# Autodesk Inventor assembly: Gripper_Design_Compliant_No_UR5
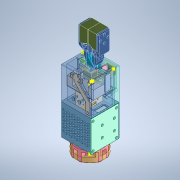
[picture p0: Inventor's stored thumbnail of the model, 180x180]
Saved by Autodesk Inventor 2022 (Build 260153000, 153)
## iProperties
Created: 2021-07-25
Part Number: Gripper_Design_Compliant_No_UR5
Document SubType Name: Assembly
Designer: exllu
Author: exllu
## Documents named in this file (27)
- C:\Users\kylem\OneDrive\Documents\1 - Documents\Gripper Design\Gripper_Design_Compliant_No_UR5.iam
- C:\Users\kylem\OneDrive\Documents\1 - Documents\Gripper Design\Motor_XM,H-430_idler.ipt
- C:\Users\kylem\OneDrive\Documents\1 - Documents\Gripper Design\Carriage_8381K550.iam
- C:\Users\kylem\OneDrive\Documents\1 - Documents\Gripper Design\Rail_8381K550.iam
- C:\Users\kylem\OneDrive\Documents\1 - Documents\Gripper Design\Pinion_2664N316.ipt
- C:\Users\kylem\OneDrive\Documents\1 - Documents\Gripper Design\Drive_shaft.ipt
- C:\Users\kylem\OneDrive\Documents\1 - Documents\Gripper Design\Motor_horn_mount.ipt
- C:\Users\kylem\OneDrive\Documents\1 - Documents\Gripper Design\Rack.iam
- C:\Users\kylem\OneDrive\Documents\1 - Documents\Gripper Design\Rail_lock_washer.ipt
- C:\Users\kylem\OneDrive\Documents\1 - Documents\Gripper Design\Rail_screws.ipt
- C:\Users\kylem\OneDrive\Documents\1 - Documents\Gripper Design\Rail_mount.ipt
- C:\Users\kylem\OneDrive\Documents\1 - Documents\Gripper Design\Front_plate.ipt
- C:\Users\kylem\OneDrive\Documents\1 - Documents\Gripper Design\Compliant_plate.ipt
- C:\Users\kylem\OneDrive\Documents\1 - Documents\Gripper Design\Finger_mount.ipt
- C:\Users\kylem\OneDrive\Documents\1 - Documents\Gripper Design\Padding.ipt
- C:\Users\kylem\OneDrive\Documents\1 - Documents\Gripper Design\UR5_Mounting_Plate.ipt
- C:\Users\kylem\OneDrive\Documents\1 - Documents\Gripper Design\Motor_UR5_mount.ipt
- C:\Users\kylem\OneDrive\Documents\1 - Documents\Gripper Design\Cover_bottom.ipt
- C:\Users\kylem\OneDrive\Documents\1 - Documents\Gripper Design\Cover_top.ipt
- C:\Users\kylem\OneDrive\Documents\1 - Documents\Gripper Design\Cover_bottom_raceway_cover.ipt
- C:\Users\kylem\OneDrive\Documents\1 - Documents\Gripper Design\U2D2 and Power Board Assembly.iam
- C:\Users\kylem\OneDrive\Documents\1 - Documents\Gripper Design\Contactile Communication Hub.ipt
- C:\Users\kylem\OneDrive\Documents\1 - Documents\Gripper Design\Electronics Box.ipt
- C:\Users\kylem\OneDrive\Documents\1 - Documents\Gripper Design\Electronics Box Lid.ipt
- C:\Users\kylem\OneDrive\Documents\1 - Documents\Gripper Design\Finger Assembly Left.iam
- C:\Users\kylem\OneDrive\Documents\1 - Documents\Gripper Design\Finger Assembly Right.iam
- C:\Users\kylem\OneDrive\Documents\1 - Documents\Gripper Design\IMU_assembly.iam
## Components (39 placed, 26 different names)
1. Motor_XM,H-430_idler:1 — Flush:1, Flush:2, Flush:3, Flush:7, Mate:15, Mate:16, Mate:29, Flush:22, Mate:65, Angle:2, Mate:223, Mate:226, Mate:262
2. Rail_8381K550:3 [sub-assembly] — Mate:3, Mate:4, Mate:5, Mate:6, Flush:7, Mate:29, Mate:30, Flush:18, Flush:19, Mate:40, Mate:41, Mate:44, Mate:45, Mate:47, Mate:55, Mate:56, Mate:57, Mate:59, Mate:61, Mate:62, Flush:25
3. Rail_8381K550:4 [sub-assembly] — Mate:1, Mate:2, Mate:7, Mate:8, Mate:30, Flush:18, Flush:19, Mate:46, Mate:63
4. Carriage_8381K550:5 [sub-assembly] — Mate:4, Mate:5, Flush:12, Flush:24, Mate:67, Mate:69
5. Carriage_8381K550:6 [sub-assembly] — Mate:1, Mate:7, Mate:89, Mate:91, Mate:233
6. Carriage_8381K550:7 [sub-assembly] — Mate:3, Mate:6, Mate:80, Mate:81, Mate:82
7. Carriage_8381K550:8 [sub-assembly] — Mate:2, Mate:8, Flush:23, Mate:87, Flush:29, Mate:88
8. Pinion_2664N316:1 — Mate:20, Mate:21, Flush:20, Tangent:1, Tangent:2, Rotation/Translation:1
9. Drive_shaft:1 — Mate:17, Mate:20, Mate:21, Mate:66, Mate:228
10. Motor_horn_mount:1 — Mate:15, Mate:16, Mate:17, Mate:64, Mate:66, Mate:227, Mate:228
11. Rack:1 [sub-assembly] — Flush:20, Tangent:1, Flush:23
12. Rack:2 [sub-assembly] — Flush:12, Tangent:2, Rotation/Translation:1, Mate:70
13. Rail_lock_washer:1 — Mate:40, Mate:41
14. Rail_lock_washer:3 — Mate:44, Mate:47, Mate:54
15. Rail_lock_washer:4 — Mate:45, Mate:46, Mate:60
16. Rail_screws:1 — Mate:60, Mate:61
17. Rail_screws:2 — Mate:54, Mate:55
18. Rail_screws:3 — Mate:58, Mate:59
19. Rail_lock_washer:5 — Mate:56, Mate:57, Mate:58
20. Rail_mount:1 — Mate:62, Mate:63, Flush:25, Mate:68, Mate:135
21. Front_plate:1 — Flush:22, Mate:64, Mate:65, Mate:68, Mate:227
22. Compliant_plate:1 — Flush:24, Mate:67, Mate:69, Mate:70, Mate:139
23. Finger_mount:1 — Mate:80, Mate:81, Mate:82, Flush:26, Flush:27, Mate:243, Mate:249, Mate:260
24. Padding:1 — Flush:26, Flush:27, Mate:139
25. Compliant_plate:2 — Mate:87, Flush:29, Mate:88
26. Padding:2 — Mate:92, Flush:30, Flush:31
27. Finger_mount:2 — Mate:89, Mate:91, Mate:92, Flush:30, Flush:31, Mate:231, Flush:53, Mate:233, Mate:259
28. UR5_Mounting_Plate:1 — Mate:129
29. Motor_UR5_mount:1 — Mate:129, Mate:254, Mate:256, Mate:258
30. Cover_bottom:1 — Mate:135, Flush:35, Mate:142, Mate:143, Flush:47, Flush:50, Mate:225, Mate:261, Mate:262
31. Cover_top:1 — Flush:35, Mate:224
32. Cover_bottom_raceway_cover:1 — Mate:142, Mate:143, Mate:261
33. U2D2 and Power Board Assembly:1 [sub-assembly] — Angle:2, Flush:49, Mate:216, Mate:218, Flush:51
34. Contactile Communication Hub:1 — Flush:47, Flush:49, Mate:220
35. Electronics Box:1 — Flush:50, Mate:216, Mate:218, Mate:219, Mate:220, Mate:223, Mate:224, Mate:225, Mate:226, Flush:51, Mate:251, Mate:253, Mate:254, Mate:255, Mate:256, Mate:258
36. Electronics Box Lid:1 — Mate:219
37. Finger Assembly Right:1 [sub-assembly] — Mate:231, Flush:53, Mate:259
38. Finger Assembly Left:1 [sub-assembly] — Mate:243, Mate:249, Mate:260
39. IMU_assembly:1 [sub-assembly] — Mate:251, Mate:253, Mate:255
## Relationships (102: Mate 75, Flush 23, Tangent 2, RelateRotateTranslate 1, Angle 1)
- Mate:1 (0.1 mm): Rail_8381K550:4 ↔ Carriage_8381K550:6
- Mate:2 (0.1 mm): Rail_8381K550:4 ↔ Carriage_8381K550:8
- Mate:3 (0.1 mm): Rail_8381K550:3 ↔ Carriage_8381K550:7
- Mate:4 (0.1 mm): Rail_8381K550:3 ↔ Carriage_8381K550:5
- Mate:5 (0.2 mm): Rail_8381K550:3 ↔ Carriage_8381K550:5
- Mate:6 (0.2 mm): Rail_8381K550:3 ↔ Carriage_8381K550:7
- Mate:7 (0.2 mm): Rail_8381K550:4 ↔ Carriage_8381K550:6
- Mate:8 (0.2 mm): Rail_8381K550:4 ↔ Carriage_8381K550:8
- Flush:1: Motor_XM,H-430_idler:1
- Flush:2: Motor_XM,H-430_idler:1
- Flush:3: Motor_XM,H-430_idler:1
- Flush:7 (-20.75 mm): Motor_XM,H-430_idler:1 ↔ Rail_8381K550:3
- Mate:15: Motor_XM,H-430_idler:1 ↔ Motor_horn_mount:1
- Mate:16: Motor_XM,H-430_idler:1 ↔ Motor_horn_mount:1
- Mate:17: Drive_shaft:1 ↔ Motor_horn_mount:1
- Mate:20: Pinion_2664N316:1 ↔ Drive_shaft:1
- Mate:21: Pinion_2664N316:1 ↔ Drive_shaft:1
- Flush:12: Carriage_8381K550:5 ↔ Rack:2
- Mate:29 (-10.75 mm): Motor_XM,H-430_idler:1 ↔ Rail_8381K550:3
- Mate:30 (1 mm): Rail_8381K550:3 ↔ Rail_8381K550:4
- Flush:18: Rail_8381K550:3 ↔ Rail_8381K550:4
- Flush:19: Rail_8381K550:3 ↔ Rail_8381K550:4
- Flush:20: Pinion_2664N316:1 ↔ Rack:1
- Mate:40: Rail_8381K550:3 ↔ Rail_lock_washer:1
- Mate:41: Rail_8381K550:3 ↔ Rail_lock_washer:1
- Mate:44: Rail_8381K550:3 ↔ Rail_lock_washer:3
- Mate:45: Rail_8381K550:3 ↔ Rail_lock_washer:4
- Mate:46: Rail_8381K550:4 ↔ Rail_lock_washer:4
- Mate:47: Rail_8381K550:3 ↔ Rail_lock_washer:3
- Mate:54: Rail_lock_washer:3 ↔ Rail_screws:2
- Mate:55: Rail_8381K550:3 ↔ Rail_screws:2
- Mate:56: Rail_8381K550:3 ↔ Rail_lock_washer:5
- Mate:57: Rail_8381K550:3 ↔ Rail_lock_washer:5
- Mate:58: Rail_screws:3 ↔ Rail_lock_washer:5
- Mate:59: Rail_8381K550:3 ↔ Rail_screws:3
- Mate:60: Rail_lock_washer:4 ↔ Rail_screws:1
- Mate:61: Rail_8381K550:3 ↔ Rail_screws:1
- Mate:62: Rail_8381K550:3 ↔ Rail_mount:1
- Mate:63: Rail_8381K550:4 ↔ Rail_mount:1
- Flush:22: Motor_XM,H-430_idler:1 ↔ Front_plate:1
- Mate:64: Motor_horn_mount:1 ↔ Front_plate:1
- Mate:65: Motor_XM,H-430_idler:1 ↔ Front_plate:1
- Tangent:1 (-1 mm): Pinion_2664N316:1 ↔ Rack:1
- Tangent:2 (-1 mm): Pinion_2664N316:1 ↔ Rack:2
- Rotation/Translation:1 [RelateRotateTranslate] (39.841 mm): Pinion_2664N316:1 ↔ Rack:2
- Mate:66: Drive_shaft:1 ↔ Motor_horn_mount:1
- Flush:23: Carriage_8381K550:8 ↔ Rack:1
- Flush:24: Carriage_8381K550:5 ↔ Compliant_plate:1
- Mate:67: Carriage_8381K550:5 ↔ Compliant_plate:1
- Flush:25: Rail_8381K550:3 ↔ Rail_mount:1
- Mate:68: Rail_mount:1 ↔ Front_plate:1
- Mate:69: Carriage_8381K550:5 ↔ Compliant_plate:1
- Mate:70: Rack:2 ↔ Compliant_plate:1
- Mate:80: Carriage_8381K550:7 ↔ Finger_mount:1
- Mate:81: Carriage_8381K550:7 ↔ Finger_mount:1
- Mate:82: Carriage_8381K550:7 ↔ Finger_mount:1
- Flush:26: Finger_mount:1 ↔ Padding:1
- Flush:27: Finger_mount:1 ↔ Padding:1
- Mate:87: Carriage_8381K550:8 ↔ Compliant_plate:2
- Flush:29: Carriage_8381K550:8 ↔ Compliant_plate:2
- Mate:88: Carriage_8381K550:8 ↔ Compliant_plate:2
- Mate:89: Carriage_8381K550:6 ↔ Finger_mount:2
- Mate:91: Carriage_8381K550:6 ↔ Finger_mount:2
- Mate:92: Padding:2 ↔ Finger_mount:2
- Flush:30: Padding:2 ↔ Finger_mount:2
- Flush:31: Padding:2 ↔ Finger_mount:2
- Mate:129: UR5_Mounting_Plate:1 ↔ Motor_UR5_mount:1
- Mate:135 (0.5 mm): Rail_mount:1 ↔ Cover_bottom:1
- Mate:139: Compliant_plate:1 ↔ Padding:1
- Flush:35: Cover_bottom:1 ↔ Cover_top:1
- Mate:142: Cover_bottom:1 ↔ Cover_bottom_raceway_cover:1
- Mate:143: Cover_bottom:1 ↔ Cover_bottom_raceway_cover:1
- Angle:2 (180 deg): Motor_XM,H-430_idler:1 ↔ U2D2 and Power Board Assembly:1
- Flush:47 (4 mm): Cover_bottom:1 ↔ Contactile Communication Hub:1
- Flush:49 (-1 mm): U2D2 and Power Board Assembly:1 ↔ Contactile Communication Hub:1
- Flush:50: Cover_bottom:1 ↔ Electronics Box:1
- Mate:216 (9 mm): U2D2 and Power Board Assembly:1 ↔ Electronics Box:1
- Mate:218 (1 mm): U2D2 and Power Board Assembly:1 ↔ Electronics Box:1
- Mate:219: Electronics Box:1 ↔ Electronics Box Lid:1
- Mate:220 (1 mm): Contactile Communication Hub:1 ↔ Electronics Box:1
- Mate:223: Motor_XM,H-430_idler:1 ↔ Electronics Box:1
- Mate:224: Cover_top:1 ↔ Electronics Box:1
- Mate:225: Cover_bottom:1 ↔ Electronics Box:1
- Mate:226: Motor_XM,H-430_idler:1 ↔ Electronics Box:1
- Flush:51 (2 mm): U2D2 and Power Board Assembly:1 ↔ Electronics Box:1
- Mate:227: Motor_horn_mount:1 ↔ Front_plate:1
- Mate:228: Drive_shaft:1 ↔ Motor_horn_mount:1
- Mate:231: Finger_mount:2 ↔ Finger Assembly Right:1
- Flush:53: Finger_mount:2 ↔ Finger Assembly Right:1
- Mate:233: Carriage_8381K550:6 ↔ Finger_mount:2
- Mate:243: Finger_mount:1 ↔ Finger Assembly Left:1
- Mate:249: Finger_mount:1 ↔ Finger Assembly Left:1
- Mate:251: Electronics Box:1 ↔ IMU_assembly:1
- Mate:253: Electronics Box:1 ↔ IMU_assembly:1
- Mate:254: Motor_UR5_mount:1 ↔ Electronics Box:1
- Mate:255: Electronics Box:1 ↔ IMU_assembly:1
- Mate:256: Motor_UR5_mount:1 ↔ Electronics Box:1
- Mate:258: Motor_UR5_mount:1 ↔ Electronics Box:1
- Mate:259: Finger_mount:2 ↔ Finger Assembly Right:1
- Mate:260: Finger_mount:1 ↔ Finger Assembly Left:1
- Mate:261 (0.5 mm): Cover_bottom:1 ↔ Cover_bottom_raceway_cover:1
- Mate:262: Motor_XM,H-430_idler:1 ↔ Cover_bottom:1
